# Autodesk Inventor assembly: Dual Extruder With Auto Leveling
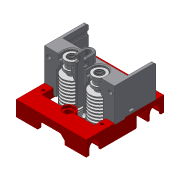
[picture p0: Inventor's stored thumbnail of the model, 180x180]
Saved by Autodesk Inventor 2015 (Build 190159000, 159)
## iProperties
Created: 2020-01-08
Part Number: Dual Extruder With Auto Leveling
Document SubType Name: Assembly
Designer: Ghassan Yusuf
Author: Ghassan Yusuf
## Documents named in this file (4)
- X:\TAKEONE\Products\takeone-3D-printer\model\3D\Dual Extruder With Auto Leveling.iam
- X:\TAKEONE\Products\takeone-3D-printer\model\3D\Carriage.ipt
- X:\TAKEONE\Products\takeone-3D-printer\model\3D\Extruder Heat Sink.ipt
- D:\Desktop\Dual Extruder Holder.ipt
## Components (4 placed, 3 different names)
1. Carriage:1 — Flush:6, Mate:1, Flush:7, Flush:8, Mate:4, Flush:9, Mate:5
2. Extruder Heat Sink:1 — Flush:1, Flush:2, Flush:4, Flush:5, Flush:8, Insert:1
3. Extruder Heat Sink:2 — Flush:1, Flush:2, Flush:4, Flush:5
4. Dual Extruder Holder:1 — Mate:4, Flush:9, Insert:1, Mate:5
## Relationships (12: Flush 8, Mate 3, Insert 1)
- Flush:1: Extruder Heat Sink:1 ↔ Extruder Heat Sink:2
- Flush:2: Extruder Heat Sink:1 ↔ Extruder Heat Sink:2
- Flush:4 (32 mm): Extruder Heat Sink:1 ↔ Extruder Heat Sink:2
- Flush:5: Extruder Heat Sink:1 ↔ Extruder Heat Sink:2
- Flush:6: Carriage:1
- Mate:1: Carriage:1
- Flush:7: Carriage:1
- Flush:8 (-20.5 mm): Carriage:1 ↔ Extruder Heat Sink:1
- Mate:4: Carriage:1 ↔ Dual Extruder Holder:1
- Flush:9: Carriage:1 ↔ Dual Extruder Holder:1
- Insert:1: Extruder Heat Sink:1 ↔ Dual Extruder Holder:1
- Mate:5: Carriage:1 ↔ Dual Extruder Holder:1
